# Autodesk Inventor assembly: PS18-16 assy
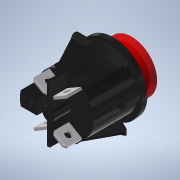
[picture p0: Inventor's stored thumbnail of the model, 180x180]
Saved by Autodesk Inventor 2022.1 (Build 261234000, 234)
## iProperties
Created: 2019-08-22
Part Number: PS18-16 assy
Material: Типовые
Document SubType Name: Assembly
Designer: Иванов Д.А.
Mass: 7.92502 g
Surface Area: 77.8703 cm^2
Volume: 5.34921 cm^3
Density: 1.48153 g/cm^3
Author: Иванов Д.А.
## Documents named in this file (4)
- E:\School\El Camino Spring 2023\Cadd 43\Group Project\Premilinary Design\PS18-16 push lached button\PS18-16 assy.iam
- E:\School\El Camino Spring 2023\Cadd 43\Group Project\Premilinary Design\PS18-16 push lached button\body.ipt
- E:\School\El Camino Spring 2023\Cadd 43\Group Project\Premilinary Design\PS18-16 push lached button\plastic diffuser.ipt
- E:\School\El Camino Spring 2023\Cadd 43\Group Project\Premilinary Design\PS18-16 push lached button\contact.ipt
## Components (3 placed, 3 different names)
1. body:1 — Вставка:1, Заподлицо:1, Совмещение:1
2. plastic diffuser:1 — Вставка:1
3. contact:1 — Заподлицо:1
## Relationships (3: Insert 1, Flush 1, Mate 1)
- Вставка:1 [Insert] (-4 mm): body:1 ↔ plastic diffuser:1
- Заподлицо:1 [Flush]: body:1 ↔ contact:1
- Совмещение:1 [Mate]: body:1
